# Autodesk Inventor assembly: machine vice Assembly
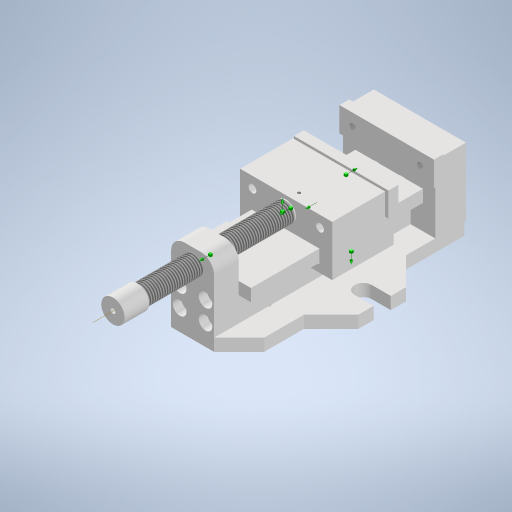
[picture p0: Inventor's stored thumbnail of the model, 512x512]
Saved by Autodesk Inventor 2023 (Build 270158000, 158)
## iProperties
Created: 2023-05-10
Part Number: machine vice Assembly
Document SubType Name: Assembly
Designer: dell
Author: dell
## Documents named in this file (10)
- D:\machine vice\machine vice Assembly.iam
- D:\machine vice\Groundplate.ipt
- D:\machine vice\Fuhrung.ipt
- D:\machine vice\Spindlesocket.ipt
- D:\machine vice\Feste Backe.ipt
- D:\machine vice\Lose Backe.ipt
- D:\machine vice\Spannbacke(n).ipt
- D:\machine vice\Trapezspindle.ipt
- D:\machine vice\Fuhrungschiene(n).ipt
- D:\machine vice\Druckhulse.ipt
## Components (11 placed, 9 different names)
1. Groundplate:1 — Mate:1, Flush:1, Mate:2, Mate:3, Flush:2
2. Spindlesocket:1 — Mate:1, Flush:1, Mate:2, Mate:4, Mate:5
3. Fuhrung:1 — Mate:3, Mate:4, Mate:5, Mate:6, Mate:7, Mate:8, Mate:12, Mate:13
4. Feste Backe:1 — Mate:6, Mate:7, Flush:2, Mate:8, Mate:10, Mate:11, Flush:3
5. Spannbacke(n):1 — Mate:10, Mate:11, Flush:3
6. Lose Backe:1 — Mate:12, Mate:13, Flush:4, Mate:15, Flush:5, Mate:16, Flush:6, Flush:7, Mate:17, Mate:18, Mate:19
7. Fuhrungschiene(n):1 — Flush:4, Mate:15, Flush:5
8. Fuhrungschiene(n):2 — Mate:16, Flush:6, Flush:7
9. Spannbacke(n):2 — Mate:17
10. Druckhulse:1 — Mate:18, Mate:19, Mate:20, Mate:21
11. Trapezspindle:1 — Mate:20, Mate:21
## Relationships (26: Mate 19, Flush 7)
- Mate:1: Groundplate:1 ↔ Spindlesocket:1
- Flush:1: Groundplate:1 ↔ Spindlesocket:1
- Mate:2: Groundplate:1 ↔ Spindlesocket:1
- Mate:3: Groundplate:1 ↔ Fuhrung:1
- Mate:4: Spindlesocket:1 ↔ Fuhrung:1
- Mate:5: Spindlesocket:1 ↔ Fuhrung:1
- Mate:6: Fuhrung:1 ↔ Feste Backe:1
- Mate:7: Fuhrung:1 ↔ Feste Backe:1
- Flush:2: Groundplate:1 ↔ Feste Backe:1
- Mate:8: Fuhrung:1 ↔ Feste Backe:1
- Mate:10: Feste Backe:1 ↔ Spannbacke(n):1
- Mate:11: Feste Backe:1 ↔ Spannbacke(n):1
- Flush:3: Feste Backe:1 ↔ Spannbacke(n):1
- Mate:12: Fuhrung:1 ↔ Lose Backe:1
- Mate:13: Fuhrung:1 ↔ Lose Backe:1
- Flush:4: Lose Backe:1 ↔ Fuhrungschiene(n):1
- Mate:15: Lose Backe:1 ↔ Fuhrungschiene(n):1
- Flush:5: Lose Backe:1 ↔ Fuhrungschiene(n):1
- Mate:16: Lose Backe:1 ↔ Fuhrungschiene(n):2
- Flush:6: Lose Backe:1 ↔ Fuhrungschiene(n):2
- Flush:7: Lose Backe:1 ↔ Fuhrungschiene(n):2
- Mate:17: Lose Backe:1 ↔ Spannbacke(n):2
- Mate:18: Lose Backe:1 ↔ Druckhulse:1
- Mate:19: Lose Backe:1 ↔ Druckhulse:1
- Mate:20: Druckhulse:1 ↔ Trapezspindle:1
- Mate:21: Druckhulse:1 ↔ Trapezspindle:1
